# Autodesk Inventor assembly: am-2566a
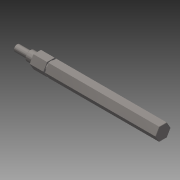
[picture p0: Inventor's stored thumbnail of the model, 180x180]
Saved by Autodesk Inventor 2018 (Build 220112000, 112)
## iProperties
Category: Toughbox Mini Kit
Company: Autodesk Inc.
Created: 2017-12-14
Part Number: am-2566a
Document SubType Name: Assembly
Designer: Autodesk Inc.
Title: am-2566a Short 500 Hex Steel Output Shaft with Magnet for Toughbox Series.STEP
Author: Autodesk Inc.
Keywords: Drive Base Kit
## Documents named in this file (3)
- D:\FIRST 2018\FIRST 2018 Inventor\FIRST 2018 Drive Base Kit\am-2566a.iam
- D:\FIRST 2018\FIRST 2018 Inventor\FIRST 2018 Drive Base Kit\Parts\sc-2566a TB Output Shaft Hex AM14U mag.ipt
- D:\FIRST 2018\FIRST 2018 Inventor\FIRST 2018 Drive Base Kit\Parts\250x1000 dowel.ipt
## Components (2 placed, 2 different names)
1. sc-2566a TB Output Shaft Hex AM14U mag_1 — Mate:1, Flush:1
2. 250x1000 dowel_2 — Mate:1, Flush:1
## Relationships (2: Mate 1, Flush 1)
- Mate:1: sc-2566a TB Output Shaft Hex AM14U mag_1 ↔ 250x1000 dowel_2
- Flush:1 (-12.7 mm): sc-2566a TB Output Shaft Hex AM14U mag_1 ↔ 250x1000 dowel_2
